# Autodesk Inventor assembly: Alpha Idler Assembly
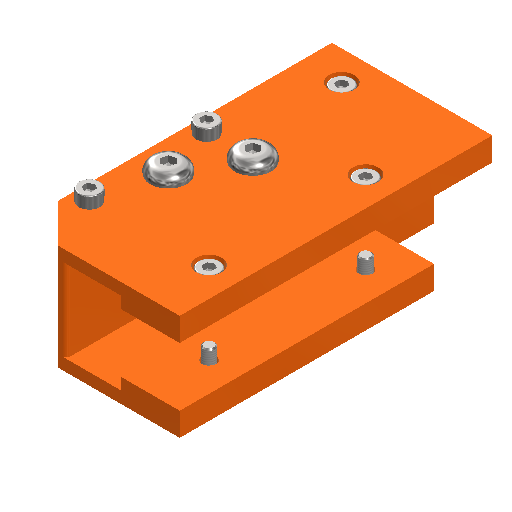
[picture p0: Inventor's stored thumbnail of the model, 512x512]
Saved by Autodesk Inventor 2023.2 (Build 272271000, 271)
## iProperties
Created: 2023-02-03
Part Number: Alpha Idler Assembly
Document SubType Name: Assembly
Designer: remop
Author: remop
## Documents named in this file (9)
- C:\Users\remop\OneDrive\Documents\Inventor\3D Printers\LuEVO\Mk5_FullKinematic\Alpha Idler Assembly.iam
- C:\Users\remop\OneDrive\Documents\Inventor\3D Printers\LuEVO\Mk5_FullKinematic\Alpha Idler Holder.ipt
- C:\Users\remop\OneDrive\Documents\Inventor\3D Printers\LuEVO\Mk5_FullKinematic\6mm toothed idler.ipt
- C:\Users\remop\OneDrive\Documents\Inventor\3D Printers\LuEVO\Mk5_FullKinematic\Alpha Idler Top.ipt
- C:\Users\remop\OneDrive\Documents\Inventor\Content Center Files\R2023\en-US\AS 1420\AS 1420 - 1973 - M3 x 6.ipt
- C:\Users\remop\OneDrive\Documents\Inventor\Content Center Files\R2023\en-US\AS 1420\AS 1420 - 1973 - M3 x 12.ipt
- C:\Users\remop\OneDrive\Documents\Inventor\3D Printers\LuEVO\Mk5_FullKinematic\Idler Spacer.ipt
- C:\Users\remop\OneDrive\Documents\Inventor\Content Center Files\R2023\en-US\BS 4168(6)\BS 4168 - M5 x 30(6).ipt
- C:\Users\remop\OneDrive\Documents\Inventor\Content Center Files\R2023\en-US\DIN 1587\DIN 1587 - M5 x 0.8.ipt
## Components (18 placed, 8 different names)
1. Alpha Idler Holder:1 — Rigid:1, Rotational:1, Flush:1, Mate:1, Flush:2, Insert:4, Insert:5, Insert:6, Rigid:3, Rigid:6, Rigid:7
2. 6mm toothed idler:1 — Rotational:1
3. 6mm toothed idler:2 — Rigid:1
4. Alpha Idler Top:1 — Flush:1, Mate:1, Flush:2, Insert:1, Insert:2, Insert:3, Insert:7, Insert:8, Rigid:2, Rigid:4, Rigid:5
5. AS 1420 - Metric M3 x 6:1 — Insert:1
6. AS 1420 - Metric M3 x 6:2 — Insert:2
7. AS 1420 - Metric M3 x 6:3 — Insert:3
8. AS 1420 - Metric M3 x 6:4 — Insert:4
9. AS 1420 - Metric M3 x 6:5 — Insert:5
10. AS 1420 - Metric M3 x 6:6 — Insert:6
11. AS 1420 - Metric M3 x 12:1 — Insert:7
12. AS 1420 - Metric M3 x 12:2 — Insert:8
13. Idler Spacer:1 — Rigid:3
14. Idler Spacer:2 — Rigid:2
15. BS 4168 : Part 6 Hexagon socket countersunk and button head screws - Metric series - Metric M5 x 30:1 — Rigid:4
16. BS 4168 : Part 6 Hexagon socket countersunk and button head screws - Metric series - Metric M5 x 30:2 — Rigid:5
17. DIN 1587 M5:1 — Rigid:6
18. DIN 1587 M5:2 — Rigid:7
## Relationships (19: Insert 8, WeldJoint 7, Flush 2, RevoluteJoint 1, Mate 1)
- Rigid:1 [WeldJoint] (-1 mm): Alpha Idler Holder:1 ↔ 6mm toothed idler:2
- Rotational:1 [RevoluteJoint] (-10 mm): Alpha Idler Holder:1 ↔ 6mm toothed idler:1
- Flush:1: Alpha Idler Holder:1 ↔ Alpha Idler Top:1
- Mate:1: Alpha Idler Holder:1 ↔ Alpha Idler Top:1
- Flush:2: Alpha Idler Holder:1 ↔ Alpha Idler Top:1
- Insert:1: Alpha Idler Top:1 ↔ AS 1420 - Metric M3 x 6:1
- Insert:2: Alpha Idler Top:1 ↔ AS 1420 - Metric M3 x 6:2
- Insert:3: Alpha Idler Top:1 ↔ AS 1420 - Metric M3 x 6:3
- Insert:4: Alpha Idler Holder:1 ↔ AS 1420 - Metric M3 x 6:4
- Insert:5: Alpha Idler Holder:1 ↔ AS 1420 - Metric M3 x 6:5
- Insert:6: Alpha Idler Holder:1 ↔ AS 1420 - Metric M3 x 6:6
- Insert:7: Alpha Idler Top:1 ↔ AS 1420 - Metric M3 x 12:1
- Insert:8: Alpha Idler Top:1 ↔ AS 1420 - Metric M3 x 12:2
- Rigid:2 [WeldJoint]: Alpha Idler Top:1 ↔ Idler Spacer:2
- Rigid:3 [WeldJoint]: Alpha Idler Holder:1 ↔ Idler Spacer:1
- Rigid:4 [WeldJoint]: Alpha Idler Top:1 ↔ BS 4168 : Part 6 Hexagon socket countersunk and button head screws - Metric series - Metric M5 x 30:1
- Rigid:5 [WeldJoint]: Alpha Idler Top:1 ↔ BS 4168 : Part 6 Hexagon socket countersunk and button head screws - Metric series - Metric M5 x 30:2
- Rigid:6 [WeldJoint]: Alpha Idler Holder:1 ↔ DIN 1587 M5:1
- Rigid:7 [WeldJoint]: Alpha Idler Holder:1 ↔ DIN 1587 M5:2
